# Autodesk Inventor assembly: Motor_asm
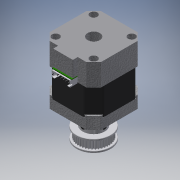
[picture p0: Inventor's stored thumbnail of the model, 180x180]
Saved by Autodesk Inventor 2019.3 (Build 233278000, 278)
## iProperties
Created: 2020-08-26
Part Number: Motor_asm
Material: Generisch
Document SubType Name: Assembly
Designer: Nicolas Frick
Author: Nicolas Frick
## Documents named in this file (3)
- C:\Users\Nicolas Frick\Sync\OneDrive\airhockeybot\mechanical_design\inventor\Motor_asm.iam
- C:\Users\Nicolas Frick\Sync\OneDrive\airhockeybot\mechanical_design\inventor\GT2 40T 5mm Bore 6mm wide pulley\GT2 40T 5 Bore v2.iam
- C:\Users\Nicolas Frick\Sync\OneDrive\airhockeybot\mechanical_design\inventor\Nema 17HS5425\Assembly1.iam
## Components (2 placed, 2 different names)
1. GT2 40T 5 Bore v2:1 [sub-assembly] — Passend:1, Passend:2
2. Assembly1:1 [sub-assembly] — Passend:1, Passend:2
## Relationships (2: Mate 2)
- Passend:1 [Mate]: GT2 40T 5 Bore v2:1 ↔ Assembly1:1
- Passend:2 [Mate]: GT2 40T 5 Bore v2:1 ↔ Assembly1:1
